# Autodesk Inventor assembly: ContinousCarriage
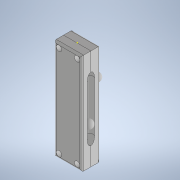
[picture p0: Inventor's stored thumbnail of the model, 180x180]
Saved by Autodesk Inventor 2022 (Build 260153000, 153)
## iProperties
Created: 2022-03-14
Part Number: ContinousCarriage
Document SubType Name: Assembly
Designer: Jorian Brusind
Author: Jorian Brusind
## Documents named in this file (3)
- C:\Users\Jorian Brusind\Documents\GitHub\HyperRail\Inventor Files\Carriage Updates\ContinousCarriage.iam
- C:\Users\Jorian Brusind\Documents\GitHub\HyperRail\Inventor Files\Carriage Updates\TestClosedLoopBearing.ipt
- C:\Users\Jorian Brusind\Documents\GitHub\HyperRail\Inventor Files\Carriage Updates\9mm_ballbearing.ipt
## Components (4 placed, 2 different names)
1. TestClosedLoopBearing:1 — Mate:1, Mate:2, Mate:3, Mate:4
2. TestClosedLoopBearing:2 — Mate:1, Mate:2, Mate:4
3. 9mm_ballbearing:1 — Mate:3
4. 9mm_ballbearing:2
## Relationships (4: Mate 4)
- Mate:1: TestClosedLoopBearing:1 ↔ TestClosedLoopBearing:2
- Mate:2: TestClosedLoopBearing:1 ↔ TestClosedLoopBearing:2
- Mate:3: TestClosedLoopBearing:1 ↔ 9mm_ballbearing:1
- Mate:4: TestClosedLoopBearing:1 ↔ TestClosedLoopBearing:2
